# Autodesk Inventor assembly: servo_plate_assembly
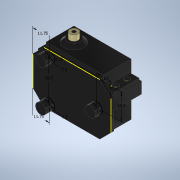
[picture p0: Inventor's stored thumbnail of the model, 180x180]
Saved by Autodesk Inventor 2020 (Build 240168000, 168)
## iProperties
Created: 2019-12-03
Part Number: servo_plate_assembly
Document SubType Name: Assembly
Designer: maste
Author: maste
## Documents named in this file (3)
- C:\Users\maste\Documents\GitHub\autobot\robot_model\servo_plate_assembly.iam
- C:\Users\maste\Documents\GitHub\autobot\robot_model\RCT-P002_servo_plate_mount.ipt
- C:\Users\maste\Documents\GitHub\autobot\robot_model\HX-15CS_15KGs_metal_gear_servo.ipt
## Components (2 placed, 2 different names)
1. RCT-P002_servo_plate_mount:1 — Mate:1, Mate:2, Mate:3
2. HX-15CS_15KGs_metal_gear_servo:1 — Mate:1, Mate:2, Mate:3
## Relationships (3: Mate 3)
- Mate:1: RCT-P002_servo_plate_mount:1 ↔ HX-15CS_15KGs_metal_gear_servo:1
- Mate:2: RCT-P002_servo_plate_mount:1 ↔ HX-15CS_15KGs_metal_gear_servo:1
- Mate:3: RCT-P002_servo_plate_mount:1 ↔ HX-15CS_15KGs_metal_gear_servo:1
